# Autodesk Inventor assembly: MK5n, A (2)
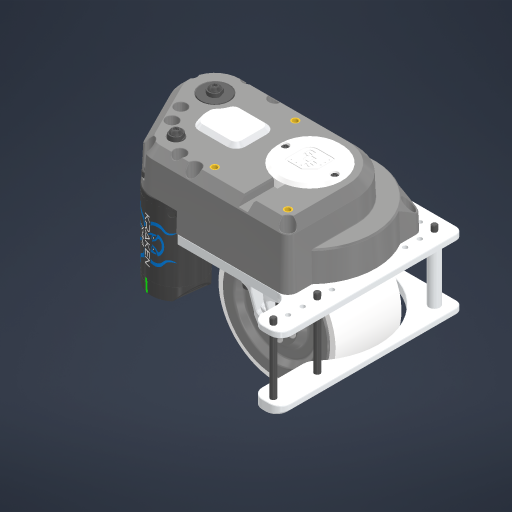
[picture p0: Inventor's stored thumbnail of the model, 512x512]
Saved by Autodesk Inventor 2024.4 (Build 284460000, 460)
## iProperties
Created: 2026-01-06
Part Number: MK5n, A (2)
Document SubType Name: Assembly
Designer: Kenji
Mass: 2676.19 g
Surface Area: 2655.27 cm^2
Volume: 1584.76 cm^3
Sending System: SOLIDWORKS 2022-2022290
MC: AMD64
MC_MODEL: Intel64 Family 6 Model 158 Stepping 10, GenuineIntel
OS: Windows_NT
FRU: Parasolid Version 33.1, build 260,  4-25-2022
FORMAT: text
GUISE: transmit
KEY: FILEMK5n, A.x_t
DATE: Fri Aug  8 12:42:24 2025
Author: Kenji
## Documents named in this file (13)
- C:\Users\Kenji\Documents\GitHub\1622-2026-Rebuilt\COTS Library\MK5N Swerve Modules\MK5n, A (2)\MK5n, A (2).iam
- C:\Users\Kenji\Documents\GitHub\1622-2026-Rebuilt\COTS Library\MK5N Swerve Modules\MK5n, A (2)\MK5n, A (2)\MK5n, A (2).ipt
- C:\Users\Kenji\Documents\GitHub\1622-2026-Rebuilt\COTS Library\MK5N Swerve Modules\MK5n, A (2)\MK5n, A (2)\MK5n, A (2)_1.ipt
- C:\Users\Kenji\Documents\GitHub\1622-2026-Rebuilt\COTS Library\MK5N Swerve Modules\MK5n, A (2)\MK5n, A (2)\MK5n, A (2)_2.ipt
- C:\Users\Kenji\Documents\GitHub\1622-2026-Rebuilt\COTS Library\MK5N Swerve Modules\MK5n, A (2)\MK5n, A (2)\MK5n, A (2)_3.ipt
- C:\Users\Kenji\Documents\GitHub\1622-2026-Rebuilt\COTS Library\MK5N Swerve Modules\MK5n, A (2)\MK5n, A (2)\MK5n, A (2)_4.ipt
- C:\Users\Kenji\Documents\GitHub\1622-2026-Rebuilt\COTS Library\MK5N Swerve Modules\MK5n, A (2)\MK5n, A (2)\MK5n, A (2)_5.ipt
- C:\Users\Kenji\Documents\GitHub\1622-2026-Rebuilt\COTS Library\MK5N Swerve Modules\MK5n, A (2)\MK5n, A (2)\MK5n, A (2)_6.ipt
- C:\Users\Kenji\Documents\GitHub\1622-2026-Rebuilt\COTS Library\MK5N Swerve Modules\MK5n, A (2)\MK5n, A (2)\MK5n, A (2)_7.ipt
- C:\Users\Kenji\Documents\GitHub\1622-2026-Rebuilt\COTS Library\MK5N Swerve Modules\MK5n, A (2)\MK5n, A (2)\MK5n, A (2)_8.ipt
- C:\Users\Kenji\Documents\GitHub\1622-2026-Rebuilt\COTS Library\MK5N Swerve Modules\MK5n, A (2)\MK5n, A (2)\MK5n, A (2)_9.ipt
- C:\Users\Kenji\Documents\GitHub\1622-2026-Rebuilt\COTS Library\Motors\COTS_WCP-0941_KrakenX44.ipt
- C:\Users\Kenji\Documents\GitHub\1622-2026-Rebuilt\COTS Library\Motors\COTS_WCP-0940_KrakenX60_New.ipt
## Components (12 placed, 12 different names)
1. MK5n, A (2) — Mate:1, Mate:2, Mate:3, Mate:4
2. MK5n, A (2)_1 — Mate:1, Mate:2, Angle:1
3. MK5n, A (2)_2 — Mate:5, Mate:8, Mate:9, Mate:10, Mate:11, Mate:12, Mate:13, Mate:14, Mate:15, Mate:16
4. MK5n, A (2)_3 — Mate:10, Mate:11
5. MK5n, A (2)_4 — Mate:12, Flush:2, Flush:3
6. MK5n, A (2)_5 — Mate:13, Flush:3, Mate:16
7. MK5n, A (2)_6 — Mate:14, Flush:1
8. MK5n, A (2)_7 — Mate:15, Flush:1, Flush:2
9. MK5n, A (2)_8 — Mate:6, Mate:7, Mate:8, Mate:9
10. MK5n, A (2)_9 — Mate:3, Mate:4, Angle:1, Mate:5, Mate:6, Mate:7, Mate:17, Mate:18, Mate:19, Mate:20, Mate:21, Mate:22
11. COTS_WCP-0941_KrakenX44:1 — Mate:20, Mate:21, Mate:22
12. COTS_WCP-0940_KrakenX60_New:1 — Mate:17, Mate:18, Mate:19
## Relationships (26: Mate 22, Flush 3, Angle 1)
- Mate:1: MK5n, A (2) ↔ MK5n, A (2)_1
- Mate:2: MK5n, A (2) ↔ MK5n, A (2)_1
- Mate:3: MK5n, A (2) ↔ MK5n, A (2)_9
- Mate:4: MK5n, A (2) ↔ MK5n, A (2)_9
- Angle:1 (0 deg): MK5n, A (2)_1 ↔ MK5n, A (2)_9
- Mate:5: MK5n, A (2)_2 ↔ MK5n, A (2)_9
- Mate:6: MK5n, A (2)_8 ↔ MK5n, A (2)_9
- Mate:7: MK5n, A (2)_8 ↔ MK5n, A (2)_9
- Mate:8: MK5n, A (2)_2 ↔ MK5n, A (2)_8
- Mate:9: MK5n, A (2)_2 ↔ MK5n, A (2)_8
- Mate:10: MK5n, A (2)_2 ↔ MK5n, A (2)_3
- Mate:11: MK5n, A (2)_2 ↔ MK5n, A (2)_3
- Mate:12: MK5n, A (2)_2 ↔ MK5n, A (2)_4
- Mate:13: MK5n, A (2)_2 ↔ MK5n, A (2)_5
- Mate:14: MK5n, A (2)_2 ↔ MK5n, A (2)_6
- Mate:15: MK5n, A (2)_2 ↔ MK5n, A (2)_7
- Flush:1: MK5n, A (2)_6 ↔ MK5n, A (2)_7
- Flush:2: MK5n, A (2)_4 ↔ MK5n, A (2)_7
- Flush:3: MK5n, A (2)_4 ↔ MK5n, A (2)_5
- Mate:16: MK5n, A (2)_2 ↔ MK5n, A (2)_5
- Mate:17: MK5n, A (2)_9 ↔ COTS_WCP-0940_KrakenX60_New:1
- Mate:18: MK5n, A (2)_9 ↔ COTS_WCP-0940_KrakenX60_New:1
- Mate:19: MK5n, A (2)_9 ↔ COTS_WCP-0940_KrakenX60_New:1
- Mate:20: MK5n, A (2)_9 ↔ COTS_WCP-0941_KrakenX44:1
- Mate:21: MK5n, A (2)_9 ↔ COTS_WCP-0941_KrakenX44:1
- Mate:22: MK5n, A (2)_9 ↔ COTS_WCP-0941_KrakenX44:1
